# Autodesk Inventor assembly: Bed
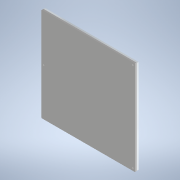
[picture p0: Inventor's stored thumbnail of the model, 180x180]
Saved by Autodesk Inventor 2020.2 (Build 242310000, 310)
## iProperties
Created: 2020-07-29
Part Number: Bed
Document SubType Name: Assembly
Designer: JK
Author: JK
## Documents named in this file (3)
- C:\Users\JK\Documents\Inventor\Anet Upgrade\Bed.iam
- C:\Users\JK\Documents\Inventor\Anet Upgrade\GlassBed.ipt
- C:\Users\JK\Documents\Inventor\Anet Upgrade\GlassBedsupport.ipt
## Components (2 placed, 2 different names)
1. GlassBed:1 — Mate:1, Flush:1, Flush:2
2. GlassBedsupport:1 — Mate:1, Flush:1, Flush:2
## Relationships (3: Flush 2, Mate 1)
- Mate:1: GlassBed:1 ↔ GlassBedsupport:1
- Flush:1: GlassBed:1 ↔ GlassBedsupport:1
- Flush:2: GlassBed:1 ↔ GlassBedsupport:1
